# Autodesk Inventor assembly: Baugruppe1
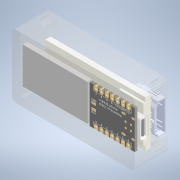
[picture p0: Inventor's stored thumbnail of the model, 180x180]
Saved by Autodesk Inventor 2022 (Build 260153000, 153)
## iProperties
Created: 2021-11-03
Part Number: Baugruppe1
Document SubType Name: Assembly
Designer: lukas
Author: lukas
## Documents named in this file (7)
- C:\Users\lukas\Dokumente\GitHub\mobileKVM\CAD\Baugruppe1.iam
- C:\Users\lukas\Dokumente\GitHub\mobileKVM\CAD\TTLUSB.ipt
- C:\Users\lukas\Dokumente\GitHub\mobileKVM\CAD\hdmi grabber.ipt
- C:\Users\lukas\Dokumente\GitHub\mobileKVM\CAD\USB-Hub.ipt
- C:\Users\lukas\Dokumente\GitHub\mobileKVM\CAD\Gehäuse.ipt
- C:\Users\lukas\Dokumente\GitHub\mobileKVM\CAD\HDMI\HDMI.ipt
- C:\Users\lukas\Dokumente\GitHub\mobileKVM\CAD\xiao\Seeeduino XIAO Arduino SW2021.ipt
## Components (6 placed, 6 different names)
1. hdmi grabber:1 — Passend:2, Passend:10, Fluchtend:8, Passend:11, Passend:16, Passend:22
2. Gehäuse:1 — Passend:2, Passend:15, Passend:16, Passend:17, Passend:21, Passend:23, Passend:24, Passend:25, Passend:26, Passend:27
3. HDMI:1 — Passend:10, Fluchtend:8, Passend:11
4. TTLUSB:2 — Passend:17, Passend:21, Passend:27
5. USB-Hub:2 — Passend:15, Passend:22, Passend:23
6. Seeeduino XIAO Arduino SW2021:1 — Passend:24, Passend:25, Passend:26
## Relationships (14: Mate 13, Flush 1)
- Passend:2 [Mate]: hdmi grabber:1 ↔ Gehäuse:1
- Passend:10 [Mate]: hdmi grabber:1 ↔ HDMI:1
- Fluchtend:8 [Flush]: hdmi grabber:1 ↔ HDMI:1
- Passend:11 [Mate]: hdmi grabber:1 ↔ HDMI:1
- Passend:15 [Mate]: Gehäuse:1 ↔ USB-Hub:2
- Passend:16 [Mate]: hdmi grabber:1 ↔ Gehäuse:1
- Passend:17 [Mate]: Gehäuse:1 ↔ TTLUSB:2
- Passend:21 [Mate]: Gehäuse:1 ↔ TTLUSB:2
- Passend:22 [Mate]: hdmi grabber:1 ↔ USB-Hub:2
- Passend:23 [Mate]: Gehäuse:1 ↔ USB-Hub:2
- Passend:24 [Mate]: Gehäuse:1 ↔ Seeeduino XIAO Arduino SW2021:1
- Passend:25 [Mate]: Gehäuse:1 ↔ Seeeduino XIAO Arduino SW2021:1
- Passend:26 [Mate]: Gehäuse:1 ↔ Seeeduino XIAO Arduino SW2021:1
- Passend:27 [Mate]: Gehäuse:1 ↔ TTLUSB:2
